# Autodesk Inventor assembly: PCBAssembly
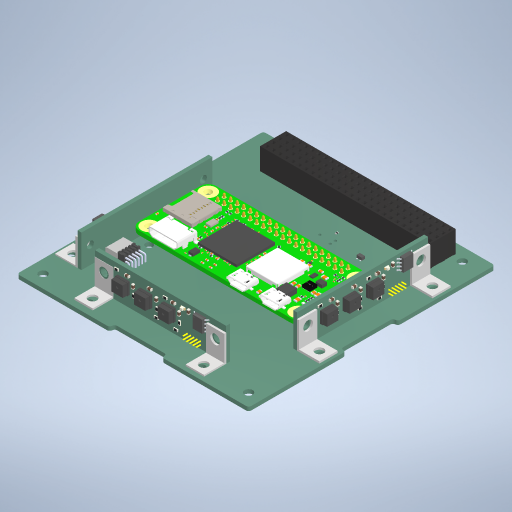
[picture p0: Inventor's stored thumbnail of the model, 512x512]
Saved by Autodesk Inventor 2023.5 (Build 275446020, 446B)
## iProperties
Created: 2026-07-20
Part Number: PCBAssembly
Document SubType Name: Assembly
Designer: User
Author: User
## Documents named in this file (5)
- C:\Users\User\Projects\missionpegasusPCB\CAD\PCBAssembly.iam
- C:\Users\User\Projects\missionpegasusPCB\CAD\615Bracket.ipt
- C:\Users\User\Projects\missionpegasusPCB\main-board\mainboard2\mainboard2.iam
- C:\Users\User\Projects\missionpegasusPCB\mezzanine-board\sensorboard3\sensorboard3.iam
- C:\Users\User\Downloads\User Library-40-pin GPIO Header for Raspberry Pi (color-coded)\User Library-40-pin GPIO Header for Raspberry Pi (color-coded).ipt
## Components (11 placed, 4 different names)
1. mainboard2:1 [sub-assembly] — Mate:1, Mate:2, Mate:4, Mate:5, Mate:7, Mate:8, Mate:9, Mate:10
2. 615Bracket:4 — Mate:3
3. sensorboard3:1 [sub-assembly] — Mate:1, Mate:2, Mate:3, Mate:4, Mate:6
4. User Library-40-pin GPIO Header for Raspberry Pi (color-coded):1 — Mate:5
5. 615Bracket:5 — Mate:6
6. sensorboard3:2 [sub-assembly] — Mate:7, Mate:8, Mate:11, Mate:12
7. sensorboard3:4 [sub-assembly] — Mate:9, Mate:10, Mate:13, Mate:14
8. 615Bracket:8 — Mate:13
9. 615Bracket:9 — Mate:14
10. 615Bracket:10 — Mate:12
11. 615Bracket:11 — Mate:11
## Relationships (14: Mate 14)
- Mate:1: mainboard2:1 ↔ sensorboard3:1
- Mate:2: mainboard2:1 ↔ sensorboard3:1
- Mate:3: 615Bracket:4 ↔ sensorboard3:1
- Mate:4: mainboard2:1 ↔ sensorboard3:1
- Mate:5: mainboard2:1 ↔ User Library-40-pin GPIO Header for Raspberry Pi (color-coded):1
- Mate:6: sensorboard3:1 ↔ 615Bracket:5
- Mate:7: mainboard2:1 ↔ sensorboard3:2
- Mate:8: mainboard2:1 ↔ sensorboard3:2
- Mate:9: mainboard2:1 ↔ sensorboard3:4
- Mate:10: mainboard2:1 ↔ sensorboard3:4
- Mate:11: sensorboard3:2 ↔ 615Bracket:11
- Mate:12: sensorboard3:2 ↔ 615Bracket:10
- Mate:13: sensorboard3:4 ↔ 615Bracket:8
- Mate:14: sensorboard3:4 ↔ 615Bracket:9
